# Autodesk Inventor assembly: PCB_LT_ICR
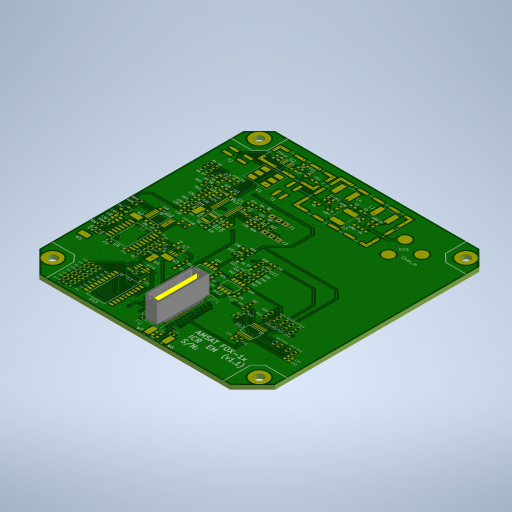
[picture p0: Inventor's stored thumbnail of the model, 512x512]
Saved by Autodesk Inventor 2023 (Build 270158000, 158)
## iProperties
Created: 2011-10-12
Part Number: PCB_LT_ICR
Document SubType Name: Assembly
Designer: Robert Davis
Description: RX PCB
Mass: 39.7863 g
Surface Area: 333.319 cm^2
Volume: 17.6679 cm^3
Density: 2.2519 g/cm^3
Author: Robert Davis
## Documents named in this file (4)
- C:\Users\User\Downloads\CAD_backup_frequent_files_20200629 (1)\PCB_LT_ICR.iam
- C:\Users\User\Downloads\CAD_backup_frequent_files_20200629 (1)\Samtec_QSH-030-01-L-D-A.ipt
- C:\Users\User\Downloads\CAD_backup_frequent_files_20200629 (1)\Samtec_QTH-030-02-L-D-A.ipt
- C:\Users\User\Downloads\CAD_backup_frequent_files_20200629 (1)\PCB_LT_ICR-EM.ipt
## Components (3 placed, 3 different names)
1. PCB_LT_ICR-EM:1 — Mate:3, Mate:4, Angle:3, Mate:1, Mate:2, Angle:4
2. Samtec_QTH-030-02-L-D-A:1 — Mate:1, Mate:2, Angle:4
3. Samtec_QSH-030-01-L-D-A:1 — Mate:3, Mate:4, Angle:3
## Relationships (6: Mate 4, Angle 2)
- Mate:3: PCB_LT_ICR-EM:1 ↔ Samtec_QSH-030-01-L-D-A:1
- Mate:4: PCB_LT_ICR-EM:1 ↔ Samtec_QSH-030-01-L-D-A:1
- Angle:3 (180 deg): PCB_LT_ICR-EM:1 ↔ Samtec_QSH-030-01-L-D-A:1
- Mate:1: PCB_LT_ICR-EM:1 ↔ Samtec_QTH-030-02-L-D-A:1
- Mate:2: PCB_LT_ICR-EM:1 ↔ Samtec_QTH-030-02-L-D-A:1
- Angle:4 (180 deg): PCB_LT_ICR-EM:1 ↔ Samtec_QTH-030-02-L-D-A:1
